# Autodesk Inventor assembly: Assembly1
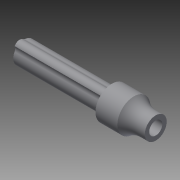
[picture p0: Inventor's stored thumbnail of the model, 180x180]
Saved by Autodesk Inventor 2015 (Build 190159000, 159)
## iProperties
Created: 2015-03-02
Part Number: Assembly1
Document SubType Name: Assembly
Designer: WASHHSST
Author: WASHHSST
## Documents named in this file (3)
- E:\JacobInventorProject\Assembly1.iam
- E:\JacobInventorProject\Part1.ipt
- E:\JacobInventorProject\Part2.ipt
## Components (2 placed, 2 different names)
1. Part1:1 — Mate:1, Mate:2, Tangent:1
2. Part2:1 — Mate:1, Mate:2, Tangent:1
## Relationships (3: Mate 2, Tangent 1)
- Mate:1: Part1:1 ↔ Part2:1
- Mate:2: Part1:1 ↔ Part2:1
- Tangent:1: Part1:1 ↔ Part2:1
